# Autodesk Inventor assembly: WheelAssembly
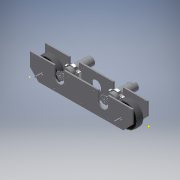
[picture p0: Inventor's stored thumbnail of the model, 180x180]
Saved by Autodesk Inventor 2017 (Build 210142000, 142)
## iProperties
Created: 2016-09-10
Part Number: WheelAssembly
Document SubType Name: Assembly
Designer: RoboticsUser
Author: RoboticsUser
## Documents named in this file (11)
- C:\Robotics\CAD\2016-17_CAD\WheelAssemble2.0.iam
- C:\Robotics\CAD\2015-16_CAD\custom cad parts\am-2648_4inWheel8mmHub.ipt
- C:\Robotics\CAD\COTSParts\Actobotics\545 parts\545556.ipt
- C:\Robotics\CAD\COTSParts\Actobotics\615 parts\615102.ipt
- C:\Robotics\CAD\COTSParts\Actobotics\634 parts\634080.ipt
- C:\Robotics\CAD\COTSParts\Motors\Andymark 2964  NeveRest 40 Motor.ipt
- C:\Users\RoboticsUser\Desktop\2015-16 CAD\COTSParts\Actobotics\615 parts\615114.ipt
- C:\Robotics\CAD\COTSParts\Tetrix\tetrix-motor-mounts-1.snapshot.1\Tetrex 2pc motor mount.ipt
- C:\Robotics\CAD\2016-17_CAD\DriveTrainPlateInside1.iam
- C:\Robotics\CAD\COTSParts\Actobotics\545 parts\545456.ipt
- C:\Robotics\CAD\2016-17_CAD\DriveTrainPlateOutside2.iam
## Components (24 placed, 10 different names)
1. am-2648_4inWheel8mmHub:2 — Mate:14, Mate:15, Mate:22
2. 545556:2 — Mate:10, Mate:11, Mate:13
3. 615102:4 — Mate:18, Mate:19, Flush:2
4. 634080:2 — Insert:70, Insert:78, Mate:10, Mate:12, Mate:15, Mate:21
5. am-2648_4inWheel8mmHub:3 — Insert:84, Insert:85
6. 545556:6 — Insert:82, Insert:83
7. 615102:5 — Insert:86, Mate:2
8. 634080:3 — Insert:66, Insert:79, Insert:82
9. Andymark 2964  NeveRest 40 Motor:2 — Insert:27, Insert:60, Mate:1, Mate:3
10. 545556:8 — Mate:1, Mate:2, Mate:4
11. 615114:2 — Insert:60
12. 615114:3
13. 545556:9 — Mate:7, Mate:18
14. Andymark 2964  NeveRest 40 Motor:3 — Mate:7, Mate:9, Flush:1, Mate:19
15. Tetrex 2pc motor mount:1 — Insert:27, Insert:80, Insert:81
16. Tetrex 2pc motor mount:2 — Mate:5, Mate:6, Mate:9, Flush:1
17. DriveTrainPlateInside1:1 [sub-assembly] — Insert:66, Insert:70, Insert:80, Insert:81, Mate:5, Mate:6, Mate:11
18. 545556:10 — Insert:87, Mate:22
19. 545456:1 — Mate:12, Mate:13, Mate:14
20. 545456:3 — Insert:83, Insert:84
21. 545556:11 — Insert:85, Insert:86
22. DriveTrainPlateOutside2:1 [sub-assembly] — Insert:78, Insert:79, Mate:23
23. 615102:6 — Mate:3, Mate:4, Mate:23
24. 615102:7 — Mate:21, Insert:87, Flush:2
## Relationships (35: Mate 19, Insert 14, Flush 2)
- Insert:27 (17.018 mm): Andymark 2964  NeveRest 40 Motor:2 ↔ Tetrex 2pc motor mount:1
- Insert:60 (16.0274 mm): Andymark 2964  NeveRest 40 Motor:2 ↔ 615114:2
- Insert:66 (-6.35 mm): 634080:3 ↔ DriveTrainPlateInside1:1
- Insert:70 (-6.35 mm): 634080:2 ↔ DriveTrainPlateInside1:1
- Insert:78 (19.05 mm): 634080:2 ↔ DriveTrainPlateOutside2:1
- Insert:79 (19.05 mm): 634080:3 ↔ DriveTrainPlateOutside2:1
- Insert:80: Tetrex 2pc motor mount:1 ↔ DriveTrainPlateInside1:1
- Insert:81: Tetrex 2pc motor mount:1 ↔ DriveTrainPlateInside1:1
- Insert:82 (12.7 mm): 545556:6 ↔ 634080:3
- Insert:83: 545556:6 ↔ 545456:3
- Insert:84: am-2648_4inWheel8mmHub:3 ↔ 545456:3
- Insert:85 (3.81 mm): am-2648_4inWheel8mmHub:3 ↔ 545556:11
- Insert:86: 615102:5 ↔ 545556:11
- Mate:1: Andymark 2964  NeveRest 40 Motor:2 ↔ 545556:8
- Mate:2: 615102:5 ↔ 545556:8
- Mate:3: Andymark 2964  NeveRest 40 Motor:2 ↔ 615102:6
- Mate:4: 545556:8 ↔ 615102:6
- Mate:5: Tetrex 2pc motor mount:2 ↔ DriveTrainPlateInside1:1
- Mate:6: Tetrex 2pc motor mount:2 ↔ DriveTrainPlateInside1:1
- Mate:7: 545556:9 ↔ Andymark 2964  NeveRest 40 Motor:3
- Mate:9: Andymark 2964  NeveRest 40 Motor:3 ↔ Tetrex 2pc motor mount:2
- Flush:1 (-17.018 mm): Andymark 2964  NeveRest 40 Motor:3 ↔ Tetrex 2pc motor mount:2
- Mate:10: 545556:2 ↔ 634080:2
- Mate:11: 545556:2 ↔ DriveTrainPlateInside1:1
- Mate:12: 634080:2 ↔ 545456:1
- Mate:13: 545556:2 ↔ 545456:1
- Mate:14: am-2648_4inWheel8mmHub:2 ↔ 545456:1
- Mate:15: am-2648_4inWheel8mmHub:2 ↔ 634080:2
- Mate:18: 615102:4 ↔ 545556:9
- Mate:19: 615102:4 ↔ Andymark 2964  NeveRest 40 Motor:3
- Mate:21: 634080:2 ↔ 615102:7
- Insert:87: 545556:10 ↔ 615102:7
- Mate:22 (3.556 mm): am-2648_4inWheel8mmHub:2 ↔ 545556:10
- Flush:2: 615102:4 ↔ 615102:7
- Mate:23 (3.81 mm): DriveTrainPlateOutside2:1 ↔ 615102:6
